# Autodesk Inventor assembly: EL2-CGB-100
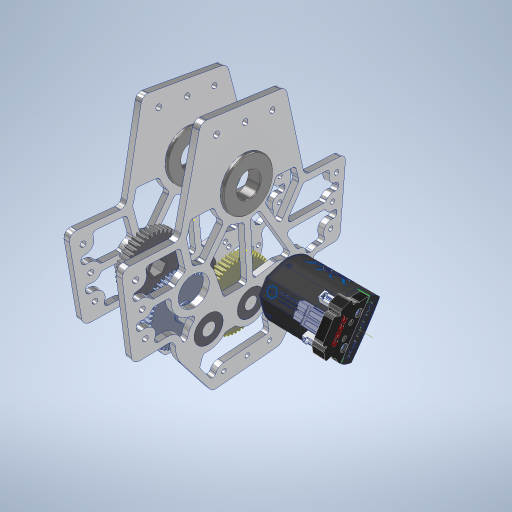
[picture p0: Inventor's stored thumbnail of the model, 512x512]
Saved by Autodesk Inventor 2023.4 (Build 274418000, 418)
## iProperties
Created: 2025-01-19
Part Number: EL2-CGB-100
Document SubType Name: Assembly
Designer: mavericks
Author: mavericks
## Documents named in this file (12)
- C:\Users\mavericks\Desktop\2025-ReefScape---CAD\Elevator\EL2-CGB\EL2-CGB-100.iam
- C:\Users\mavericks\Desktop\2025-ReefScape---CAD\Elevator\EL2-CGB\EL2-CGB-001.ipt
- C:\Users\mavericks\Desktop\2025-ReefScape---CAD\COMMON PARTS\MOTORS\Kracken with Cover and Boards.iam
- C:\Users\mavericks\Desktop\2025-ReefScape---CAD\COMMON PARTS\GEARS\WCP-1006\WCP-1006.ipt
- C:\Users\mavericks\Desktop\2025-ReefScape---CAD\COMMON PARTS\GEARS\20dp .5 hex\54t_Aluminum_Spur_Gear_20_DP_1_2_Hex_Bore_217-3573.ipt
- C:\Users\mavericks\Desktop\2025-ReefScape---CAD\COMMON PARTS\GEARS\20dp .5 hex\50t_Aluminum_Spur_Gear_20_DP_1_2_Hex_Bore_217-3572.ipt
- C:\Users\mavericks\Desktop\2025-ReefScape---CAD\COMMON PARTS\GEARS\20dp .5 hex\18t_Aluminum_Spur_Gear_20_DP_1_2_Hex_Bore_217-3209.ipt
- C:\Users\mavericks\Desktop\2025-ReefScape---CAD\COMMON PARTS\BEARINGS\0_875_ID_x_1_875_OD_X_0_500_Radial_Bearing_EE11S-2RS.ipt
- C:\Users\mavericks\Desktop\2025-ReefScape---CAD\COMMON PARTS\BEARINGS\0_500_ID_x_1_125_OD_x_0_313_WD_Flanged_Bearing_217-2731.ipt
- C:\Users\mavericks\Desktop\2025-ReefScape---CAD\COMMON PARTS\GEARS\20dp .5 hex\44t_Aluminum_Spur_Gear_20_DP_1_2_Hex_Bore_217-2710.ipt
- C:\Users\mavericks\Desktop\2025-ReefScape---CAD\COMMON PARTS\GEARS\20dp .5 hex\24t_Aluminum_Spur_Gear_20_DP_1_2_Hex_Bore_217-2704.ipt
- C:\Users\mavericks\Desktop\2025-ReefScape---CAD\Elevator\EL2-CGB\EL2-CGB-002.ipt
## Components (18 placed, 11 different names)
1. EL2-CGB-001:1 — Insert:1, Insert:2, Mate:1, Mate:2, Mate:3, Mate:6, Mate:13, Flush:2, Insert:6, Insert:7
2. Kracken with Cover and Boards:1 [sub-assembly] — Insert:1, Insert:2, Mate:4, Mate:5
3. EL2-CGB-001:2 — Mate:1, Mate:2, Mate:3, Mate:8, Mate:9, Mate:12, Flush:1, Insert:3, Insert:4, Insert:5
4. WCP-1006:1 — Mate:4, Mate:5
5. 54t_Aluminum_Spur_Gear_20_DP_1_2_Hex_Bore_217-3573:1 — Mate:6, Mate:14, Mate:15
6. 50t_Aluminum_Spur_Gear_20_DP_1_2_Hex_Bore_217-3572:1 — Mate:8, Flush:3, Mate:16
7. 24t_Aluminum_Spur_Gear_20_DP_1_2_Hex_Bore_217-2704:1 — Mate:16, Flush:4
8. 18t_Aluminum_Spur_Gear_20_DP_1_2_Hex_Bore_217-3209:1 — Mate:9, Mate:15, Flush:3
9. 44t_Aluminum_Spur_Gear_20_DP_1_2_Hex_Bore_217-2710:1 — Flush:4
10. 0_875_ID_x_1_875_OD_X_0_500_Radial_Bearing_EE11S-2RS:1 — Mate:13, Flush:2
11. 0_875_ID_x_1_875_OD_X_0_500_Radial_Bearing_EE11S-2RS:2 — Mate:12, Flush:1
12. 0_500_ID_x_1_125_OD_x_0_313_WD_Flanged_Bearing_217-2731:1 — Insert:4
13. 0_500_ID_x_1_125_OD_x_0_313_WD_Flanged_Bearing_217-2731:2 — Insert:5
14. 0_500_ID_x_1_125_OD_x_0_313_WD_Flanged_Bearing_217-2731:3 — Insert:3, Insert:9
15. 0_500_ID_x_1_125_OD_x_0_313_WD_Flanged_Bearing_217-2731:4 — Insert:7, Mate:14
16. 0_500_ID_x_1_125_OD_x_0_313_WD_Flanged_Bearing_217-2731:5 — Insert:6, Insert:8
17. EL2-CGB-002:1 — Insert:8
18. EL2-CGB-002:2 — Insert:9
## Relationships (28: Mate 15, Insert 9, Flush 4)
- Insert:1: EL2-CGB-001:1 ↔ Kracken with Cover and Boards:1
- Insert:2: EL2-CGB-001:1 ↔ Kracken with Cover and Boards:1
- Mate:1: EL2-CGB-001:1 ↔ EL2-CGB-001:2
- Mate:2 (50.8 mm): EL2-CGB-001:1 ↔ EL2-CGB-001:2
- Mate:3: EL2-CGB-001:1 ↔ EL2-CGB-001:2
- Mate:4: Kracken with Cover and Boards:1 ↔ WCP-1006:1
- Mate:5 (3.175 mm): Kracken with Cover and Boards:1 ↔ WCP-1006:1
- Mate:6: EL2-CGB-001:1 ↔ 54t_Aluminum_Spur_Gear_20_DP_1_2_Hex_Bore_217-3573:1
- Mate:8: EL2-CGB-001:2 ↔ 50t_Aluminum_Spur_Gear_20_DP_1_2_Hex_Bore_217-3572:1
- Mate:9: EL2-CGB-001:2 ↔ 18t_Aluminum_Spur_Gear_20_DP_1_2_Hex_Bore_217-3209:1
- [Mate]: EL2-CGB-001:1 ↔ 24t_Aluminum_Spur_Gear_20_DP_1_2_Hex_Bore_217-2704:1
- [Mate]: EL2-CGB-001:2 ↔ 44t_Aluminum_Spur_Gear_20_DP_1_2_Hex_Bore_217-2710:1
- Mate:12: EL2-CGB-001:2 ↔ 0_875_ID_x_1_875_OD_X_0_500_Radial_Bearing_EE11S-2RS:2
- Mate:13: EL2-CGB-001:1 ↔ 0_875_ID_x_1_875_OD_X_0_500_Radial_Bearing_EE11S-2RS:1
- Flush:1 (-3.175 mm): EL2-CGB-001:2 ↔ 0_875_ID_x_1_875_OD_X_0_500_Radial_Bearing_EE11S-2RS:2
- Flush:2 (-3.175 mm): EL2-CGB-001:1 ↔ 0_875_ID_x_1_875_OD_X_0_500_Radial_Bearing_EE11S-2RS:1
- Insert:3: EL2-CGB-001:2 ↔ 0_500_ID_x_1_125_OD_x_0_313_WD_Flanged_Bearing_217-2731:3
- Insert:4: EL2-CGB-001:2 ↔ 0_500_ID_x_1_125_OD_x_0_313_WD_Flanged_Bearing_217-2731:1
- Insert:5: EL2-CGB-001:2 ↔ 0_500_ID_x_1_125_OD_x_0_313_WD_Flanged_Bearing_217-2731:2
- Insert:6: EL2-CGB-001:1 ↔ 0_500_ID_x_1_125_OD_x_0_313_WD_Flanged_Bearing_217-2731:5
- Insert:7: EL2-CGB-001:1 ↔ 0_500_ID_x_1_125_OD_x_0_313_WD_Flanged_Bearing_217-2731:4
- Insert:8: 0_500_ID_x_1_125_OD_x_0_313_WD_Flanged_Bearing_217-2731:5 ↔ EL2-CGB-002:1
- Insert:9: 0_500_ID_x_1_125_OD_x_0_313_WD_Flanged_Bearing_217-2731:3 ↔ EL2-CGB-002:2
- Mate:14 (3.175 mm): 54t_Aluminum_Spur_Gear_20_DP_1_2_Hex_Bore_217-3573:1 ↔ 0_500_ID_x_1_125_OD_x_0_313_WD_Flanged_Bearing_217-2731:4
- Mate:15 (3.175 mm): 54t_Aluminum_Spur_Gear_20_DP_1_2_Hex_Bore_217-3573:1 ↔ 18t_Aluminum_Spur_Gear_20_DP_1_2_Hex_Bore_217-3209:1
- Flush:3: 50t_Aluminum_Spur_Gear_20_DP_1_2_Hex_Bore_217-3572:1 ↔ 18t_Aluminum_Spur_Gear_20_DP_1_2_Hex_Bore_217-3209:1
- Mate:16: 50t_Aluminum_Spur_Gear_20_DP_1_2_Hex_Bore_217-3572:1 ↔ 24t_Aluminum_Spur_Gear_20_DP_1_2_Hex_Bore_217-2704:1
- Flush:4: 24t_Aluminum_Spur_Gear_20_DP_1_2_Hex_Bore_217-2704:1 ↔ 44t_Aluminum_Spur_Gear_20_DP_1_2_Hex_Bore_217-2710:1
